# Autodesk Inventor assembly: ModulKolaNapinajacego
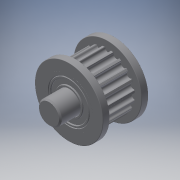
[picture p0: Inventor's stored thumbnail of the model, 180x180]
Saved by Autodesk Inventor 2019 (Build 230136000, 136)
## iProperties
Created: 2020-05-23
Part Number: ModulKolaNapinajacego
Document SubType Name: Assembly
Designer: estee
Author: estee
## Documents named in this file (3)
- C:\Users\estee\OneDrive\Pulpit\estere\1\MUM\projejt\ModulKolaNapinajacego.iam
- C:\Users\estee\OneDrive\Pulpit\estere\1\MUM\projejt\kololozyskowane\Gates_2GT_20T_Toothed.iam
- C:\Users\estee\OneDrive\Pulpit\estere\1\MUM\projejt\walekpodkolonapinajace.ipt
## Components (2 placed, 2 different names)
1. Gates_2GT_20T_Toothed:1 [sub-assembly] — Mate:1
2. walekpodkolonapinajace:1 — Mate:1
## Relationships (1: Mate 1)
- Mate:1: Gates_2GT_20T_Toothed:1 ↔ walekpodkolonapinajace:1
